# Autodesk Inventor assembly: System_ohne_Grundplatte_rechts
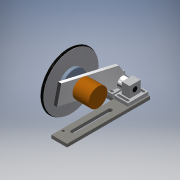
[picture p0: Inventor's stored thumbnail of the model, 180x180]
Saved by Autodesk Inventor 2017 (Build 210142000, 142)
## iProperties
Created: 2017-11-10
Part Number: System_ohne_Grundplatte_rechts
Document SubType Name: Assembly
Designer: Christoph Soppa
Author: Christoph Soppa
## Documents named in this file (9)
- C:\Users\Nils\Documents\GitHub\Eurobot2018\Hardware\Roboterplatform\Odometrie\System_ohne_Grundplatte_rechts.iam
- C:\Users\Nils\Documents\GitHub\Eurobot2018\Hardware\Roboterplatform\Odometrie\O Ring 72x3,5x65.ipt
- C:\Users\Nils\Documents\GitHub\Eurobot2018\Hardware\Roboterplatform\Odometrie\Rad d72 b4 r3.5.ipt
- C:\Users\Nils\Documents\GitHub\Eurobot2018\Hardware\Roboterplatform\Odometrie\Drehgeber 2400 .ipt
- C:\Users\Nils\Documents\GitHub\Eurobot2018\Hardware\Roboterplatform\Odometrie\Montageplatte.ipt
- C:\Users\Nils\Documents\GitHub\Eurobot2018\Hardware\Roboterplatform\Odometrie\Stehlager 6mm.ipt
- C:\Users\Nils\Documents\GitHub\Eurobot2018\Hardware\Roboterplatform\Odometrie\6mm Welle.ipt
- C:\Users\Nils\Documents\GitHub\Eurobot2018\Hardware\Roboterplatform\Odometrie\Kupplung.ipt
- C:\Users\Nils\Documents\GitHub\Eurobot2018\Hardware\Roboterplatform\Odometrie\Armrechts.ipt
## Components (9 placed, 8 different names)
1. O Ring 72x3,5x65:2 — Passend:3, Passend:4
2. Rad d72 b4 r3.5:1 — Passend:3, Passend:4, Passend:24, Passend:25
3. Drehgeber 2400 :2 — Passend:20, Passend:21, Passend:22, Passend:23
4. Montageplatte:1 — Passend:13, Fluchtend:5, Passend:14, Fluchtend:6, Fluchtend:7, Fluchtend:9, Fluchtend:10, Fluchtend:11
5. Stehlager 6mm:1 — Passend:13, Fluchtend:5, Passend:19
6. Stehlager 6mm:2 — Passend:14, Fluchtend:6, Fluchtend:7, Fluchtend:8, Passend:15, Passend:17
7. 6mm Welle:1 — Fluchtend:8, Passend:15, Passend:18
8. Kupplung:1 — Passend:22, Passend:23, Passend:24, Passend:25
9. Armrechts:1 — Passend:17, Passend:18, Passend:19, Passend:20, Passend:21
## Relationships (21: Mate 14, Flush 7)
- Passend:3 [Mate]: O Ring 72x3,5x65:2 ↔ Rad d72 b4 r3.5:1
- Passend:4 [Mate]: O Ring 72x3,5x65:2 ↔ Rad d72 b4 r3.5:1
- Passend:13 [Mate]: Montageplatte:1 ↔ Stehlager 6mm:1
- Fluchtend:5 [Flush]: Montageplatte:1 ↔ Stehlager 6mm:1
- Passend:14 [Mate]: Montageplatte:1 ↔ Stehlager 6mm:2
- Fluchtend:6 [Flush]: Montageplatte:1 ↔ Stehlager 6mm:2
- Fluchtend:7 [Flush]: Montageplatte:1 ↔ Stehlager 6mm:2
- Fluchtend:8 [Flush]: Stehlager 6mm:2 ↔ 6mm Welle:1
- Passend:15 [Mate]: Stehlager 6mm:2 ↔ 6mm Welle:1
- Passend:17 [Mate]: Stehlager 6mm:2 ↔ Armrechts:1
- Passend:18 [Mate]: 6mm Welle:1 ↔ Armrechts:1
- Passend:19 [Mate]: Stehlager 6mm:1 ↔ Armrechts:1
- Passend:20 [Mate]: Drehgeber 2400 :2 ↔ Armrechts:1
- Passend:21 [Mate]: Drehgeber 2400 :2 ↔ Armrechts:1
- Passend:22 [Mate]: Drehgeber 2400 :2 ↔ Kupplung:1
- Passend:23 [Mate]: Drehgeber 2400 :2 ↔ Kupplung:1
- Passend:24 [Mate]: Rad d72 b4 r3.5:1 ↔ Kupplung:1
- Passend:25 [Mate]: Rad d72 b4 r3.5:1 ↔ Kupplung:1
- Fluchtend:9 [Flush]: Montageplatte:1
- Fluchtend:10 [Flush]: Montageplatte:1
- Fluchtend:11 [Flush]: Montageplatte:1
